# Autodesk Inventor assembly: Marina - simplificacion
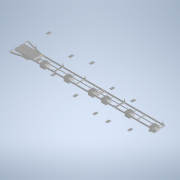
[picture p0: Inventor's stored thumbnail of the model, 180x180]
Saved by Autodesk Inventor 2022 (Build 260153000, 153)
## iProperties
Created: 2022-11-23
Part Number: Marina - simplificacion
Document SubType Name: Assembly
Designer: Maestria 1
Author: Maestria 1
## Documents named in this file (3)
- C:\Users\Maestria 1\Documents\MIMM - Francisca Cárdenas\Modelos Orza SpA\Marina - simplificacion.iam
- C:\Users\Maestria 1\Documents\MIMM - Francisca Cárdenas\Modelos Orza SpA\armazon.ipt
- C:\Users\Maestria 1\Documents\MIMM - Francisca Cárdenas\Modelos Orza SpA\peldaño.ipt
## Components (27 placed, 2 different names)
1. armazon:1 — Nivelación:1, Coincidencia:1, Coincidencia:2, Nivelación:2, Coincidencia:3, Coincidencia:4, Coincidencia:5, Nivelación:3, Coincidencia:6
2. peldaño:3
3. peldaño:4 — Coincidencia:5, Nivelación:3, Coincidencia:6
4. peldaño:5
5. peldaño:6
6. peldaño:7
7. peldaño:8
8. peldaño:9
9. peldaño:10
10. peldaño:11
11. peldaño:12
12. peldaño:13
13. peldaño:14
14. peldaño:2 — Nivelación:1, Coincidencia:1, Coincidencia:2
15. peldaño:1 — Nivelación:2, Coincidencia:3, Coincidencia:4
16. peldaño:15
17. peldaño:16
18. peldaño:17
19. peldaño:18
20. peldaño:19
21. peldaño:20
22. peldaño:21
23. peldaño:22
24. peldaño:23
25. peldaño:24
26. peldaño:25
27. peldaño:26
## Component patterns: (7 elements, first: peldaño:2 + peldaño:1)
## Relationships (9: Mate 6, Flush 3)
- Nivelación:1 [Flush]: armazon:1 ↔ peldaño:2
- Coincidencia:1 [Mate]: armazon:1 ↔ peldaño:2
- Coincidencia:2 [Mate] (25 mm): armazon:1 ↔ peldaño:2
- Nivelación:2 [Flush]: armazon:1 ↔ peldaño:1
- Coincidencia:3 [Mate]: armazon:1 ↔ peldaño:1
- Coincidencia:4 [Mate] (25 mm): armazon:1 ↔ peldaño:1
- Coincidencia:5 [Mate]: armazon:1 ↔ peldaño:4
- Nivelación:3 [Flush]: armazon:1 ↔ peldaño:4
- Coincidencia:6 [Mate] (25 mm): armazon:1 ↔ peldaño:4
